# Autodesk Inventor assembly: assembly
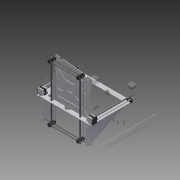
[picture p0: Inventor's stored thumbnail of the model, 180x180]
Saved by Autodesk Inventor 2013 (Build 170138000, 138)
## iProperties
Created: 2013-11-17
Part Number: assembly
Document SubType Name: Assembly
Designer: Masta
Author: Masta
## Documents named in this file (23)
- D:\prusa i3\assembly\prusa_i3plus.iam
- D:\prusa i3\assembly\lasercut_aluminium\caddy.ipt
- D:\prusa i3\assembly\lasercut_aluminium\main_frame.ipt
- D:\prusa i3\assembly\lasercut_aluminium\side_frame.ipt
- D:\prusa i3\assembly\other\fi8x320.ipt
- D:\prusa i3\assembly\other\fi8x500.ipt
- D:\prusa i3\assembly\other\M5x300.ipt
- D:\prusa i3\assembly\other\M10x530.ipt
- D:\prusa i3\assembly\plastics\Y_corner.ipt
- D:\prusa i3\assembly\other\M8x290.ipt
- D:\prusa i3\assembly\other\M8x410.ipt
- D:\prusa i3\assembly\other\LM08UU.ipt
- D:\prusa i3\assembly\plastics\Prusa_i3_X_Carriage_Belt_Clamp.ipt
- D:\prusa i3\assembly\plastics\Prusa_i3_Y_Idler.ipt
- D:\prusa i3\assembly\plastics\Z_bottom.ipt
- D:\prusa i3\assembly\plastics\Z_bottom2.ipt
- D:\prusa i3\assembly\plastics\Z_top.ipt
- D:\prusa i3\assembly\plastics\Z_top2.ipt
- D:\prusa i3\assembly\other\nema17.ipt
- D:\prusa i3\assembly\other\T10x2 330mm.ipt
- D:\prusa i3\assembly\other\T10x2 nakretka.ipt
- D:\prusa i3\assembly\plastics\X_left.ipt
- D:\prusa i3\assembly\lasercut_aluminium\stolik.ipt
## Components (48 placed, 22 different names)
1. main_frame:1 — Mate:1, Flush:3, Mate:2, Mate:3, Insert:1, Insert:2, Mate:12, Mate:14, Insert:6, Insert:7, Insert:9, Insert:10, Insert:12, Insert:13, Insert:14, Insert:15, Angle:6
2. caddy:1 — Tangent:26, Mate:9, Tangent:27, Tangent:30, Tangent:31, Mate:10, Tangent:32, Tangent:33, Mate:11, Mate:12, Mate:15, Insert:23, Insert:24
3. side_frame:1 — Flush:1, Flush:2, Flush:3, Mate:3, Flush:9
4. side_frame:2 — Flush:1, Mate:1, Flush:2, Mate:2
5. fi8x320:1 — Insert:11
6. fi8x320:2 — Insert:8
7. fi8x500:1 — Tangent:18, Tangent:19, Mate:7, Mate:8
8. fi8x500:2 — Tangent:16, Tangent:17, Mate:5, Mate:6
9. fi8x500:3
10. fi8x500:4
11. M5x300:1
12. M5x300:2
13. M10x530:1 — Insert:1, Tangent:10, Tangent:11, Tangent:12, Tangent:13, Flush:7
14. M10x530:2 — Insert:2, Tangent:8, Tangent:9, Tangent:14, Tangent:15
15. Y_corner:1 — Tangent:6, Angle:2, Tangent:12, Tangent:13, Tangent:18, Tangent:19, Mate:7, Flush:6, Flush:7, Angle:5
16. Y_corner:2 — Tangent:5, Flush:5, Tangent:7, Angle:1, Tangent:14, Tangent:15, Tangent:16, Tangent:17, Mate:5, Flush:6, Tangent:20, Tangent:21
17. Y_corner:3 — Angle:4, Tangent:10, Tangent:11, Mate:8, Mate:15
18. Y_corner:4 — Angle:3, Tangent:8, Tangent:9, Mate:6, Tangent:22, Tangent:23, Tangent:24, Tangent:25
19. M8x290:1 — Tangent:5, Tangent:6, Flush:5, Tangent:7, Flush:8, Tangent:28, Tangent:29
20. M8x290:2 — Tangent:24, Tangent:25, Flush:10
21. M8x290:3 — Tangent:20, Tangent:21, Flush:8, Flush:10
22. M8x410:1 — Tangent:22, Tangent:23, Flush:9
23. LM08UU:1
24. LM08UU:2
25. LM08UU:3 — Tangent:26, Mate:9, Tangent:27
26. LM08UU:4 — Tangent:35, Mate:17, Insert:22
27. LM08UU:5
28. LM08UU:6 — Tangent:32, Tangent:33, Mate:11
29. LM08UU:7
30. LM08UU:8
31. LM08UU:9 — Tangent:34, Mate:16
32. LM08UU:10 — Tangent:30, Tangent:31, Mate:10
33. Prusa_i3_X_Carriage_Belt_Clamp:1
34. Prusa_i3_Y_Idler:1 — Tangent:28, Tangent:29, Angle:5
35. Z_bottom:1 — Insert:6, Insert:7, Insert:8, Insert:16, Insert:17, Insert:22
36. Z_bottom2:1 — Insert:9, Insert:10, Insert:11, Insert:18, Insert:19
37. Z_top:1 — Insert:12, Insert:13
38. Z_top2:1 — Insert:14, Insert:15
39. nema17:1 — Insert:16, Insert:17, Insert:20
40. nema17:2
41. nema17:3 — Insert:18, Insert:19, Insert:21
42. nema17:4
43. T10x2 330mm:1 — Insert:20, Tangent:36
44. T10x2 330mm:2 — Insert:21
45. T10x2 nakretka:1 — Tangent:36, Mate:18, Mate:19, Mate:20
46. T10x2 nakretka:2
47. X_left:1 — Tangent:34, Mate:16, Tangent:35, Mate:17, Mate:18, Mate:19, Angle:6, Mate:20
48. stolik:1 — Insert:23, Insert:24
## Relationships (86: Tangent 32, Insert 21, Mate 18, Flush 9, Angle 6)
- Flush:1: side_frame:1 ↔ side_frame:2
- Mate:1: main_frame:1 ↔ side_frame:2
- Flush:2: side_frame:1 ↔ side_frame:2
- Flush:3: main_frame:1 ↔ side_frame:1
- Mate:2 (0.25 mm): main_frame:1 ↔ side_frame:2
- Mate:3 (0.25 mm): main_frame:1 ↔ side_frame:1
- Insert:1 (-200 mm): main_frame:1 ↔ M10x530:1
- Insert:2 (-200 mm): main_frame:1 ↔ M10x530:2
- Tangent:5: Y_corner:2 ↔ M8x290:1
- Tangent:6: Y_corner:1 ↔ M8x290:1
- Flush:5 (-11 mm): Y_corner:2 ↔ M8x290:1
- Tangent:7: Y_corner:2 ↔ M8x290:1
- Angle:1 (0 deg): Y_corner:2
- Angle:2 (0 deg): Y_corner:1
- Angle:3 (180 deg): Y_corner:4
- Angle:4 (0 deg): Y_corner:3
- Tangent:8: M10x530:2 ↔ Y_corner:4
- Tangent:9: M10x530:2 ↔ Y_corner:4
- Tangent:10: M10x530:1 ↔ Y_corner:3
- Tangent:11: M10x530:1 ↔ Y_corner:3
- Tangent:12: M10x530:1 ↔ Y_corner:1
- Tangent:13: M10x530:1 ↔ Y_corner:1
- Tangent:14: M10x530:2 ↔ Y_corner:2
- Tangent:15: M10x530:2 ↔ Y_corner:2
- Tangent:16: fi8x500:2 ↔ Y_corner:2
- Tangent:17: fi8x500:2 ↔ Y_corner:2
- Mate:5: fi8x500:2 ↔ Y_corner:2
- Mate:6: fi8x500:2 ↔ Y_corner:4
- Tangent:18: fi8x500:1 ↔ Y_corner:1
- Tangent:19: fi8x500:1 ↔ Y_corner:1
- Mate:7: fi8x500:1 ↔ Y_corner:1
- Mate:8: fi8x500:1 ↔ Y_corner:3
- Flush:6: Y_corner:1 ↔ Y_corner:2
- Flush:7 (13 mm): M10x530:1 ↔ Y_corner:1
- Tangent:20: Y_corner:2 ↔ M8x290:3
- Tangent:21: Y_corner:2 ↔ M8x290:3
- Flush:8: M8x290:1 ↔ M8x290:3
- Tangent:22: Y_corner:4 ↔ M8x410:1
- Tangent:23: Y_corner:4 ↔ M8x410:1
- Flush:9 (-11 mm): side_frame:1 ↔ M8x410:1
- Tangent:24: Y_corner:4 ↔ M8x290:2
- Tangent:25: Y_corner:4 ↔ M8x290:2
- Flush:10: M8x290:2 ↔ M8x290:3
- Tangent:26: caddy:1 ↔ LM08UU:3
- Mate:9: caddy:1 ↔ LM08UU:3
- Tangent:27: caddy:1 ↔ LM08UU:3
- Tangent:28: M8x290:1 ↔ Prusa_i3_Y_Idler:1
- Tangent:29: M8x290:1 ↔ Prusa_i3_Y_Idler:1
- Angle:5 (0 deg): Y_corner:1 ↔ Prusa_i3_Y_Idler:1
- Tangent:30: caddy:1 ↔ LM08UU:10
- Tangent:31: caddy:1 ↔ LM08UU:10
- Mate:10: caddy:1 ↔ LM08UU:10
- Tangent:32: caddy:1 ↔ LM08UU:6
- Tangent:33: caddy:1 ↔ LM08UU:6
- Mate:11: caddy:1 ↔ LM08UU:6
- Mate:12 (16.5 mm): main_frame:1 ↔ caddy:1
- Mate:14: main_frame:1
- Mate:15 (340 mm): caddy:1 ↔ Y_corner:3
- Insert:6: main_frame:1 ↔ Z_bottom:1
- Insert:7: main_frame:1 ↔ Z_bottom:1
- Insert:8: fi8x320:2 ↔ Z_bottom:1
- Insert:9: main_frame:1 ↔ Z_bottom2:1
- Insert:10: main_frame:1 ↔ Z_bottom2:1
- Insert:11: fi8x320:1 ↔ Z_bottom2:1
- Insert:12: main_frame:1 ↔ Z_top:1
- Insert:13: main_frame:1 ↔ Z_top:1
- Insert:14: main_frame:1 ↔ Z_top2:1
- Insert:15: main_frame:1 ↔ Z_top2:1
- Insert:16: Z_bottom:1 ↔ nema17:1
- Insert:17: Z_bottom:1 ↔ nema17:1
- Insert:18: Z_bottom2:1 ↔ nema17:3
- Insert:19: Z_bottom2:1 ↔ nema17:3
- Insert:20: nema17:1 ↔ T10x2 330mm:1
- Insert:21: nema17:3 ↔ T10x2 330mm:2
- Tangent:34: LM08UU:9 ↔ X_left:1
- Mate:16: LM08UU:9 ↔ X_left:1
- Tangent:35: LM08UU:4 ↔ X_left:1
- Mate:17: LM08UU:4 ↔ X_left:1
- Insert:22: LM08UU:4 ↔ Z_bottom:1
- Tangent:36: T10x2 330mm:1 ↔ T10x2 nakretka:1
- Mate:18: T10x2 nakretka:1 ↔ X_left:1
- Mate:19: T10x2 nakretka:1 ↔ X_left:1
- Angle:6 (180 deg): main_frame:1 ↔ X_left:1
- Mate:20: T10x2 nakretka:1 ↔ X_left:1
- Insert:23 (10 mm): caddy:1 ↔ stolik:1
- Insert:24 (10 mm): caddy:1 ↔ stolik:1
